# Autodesk Inventor assembly: KND-2000 Collector 01
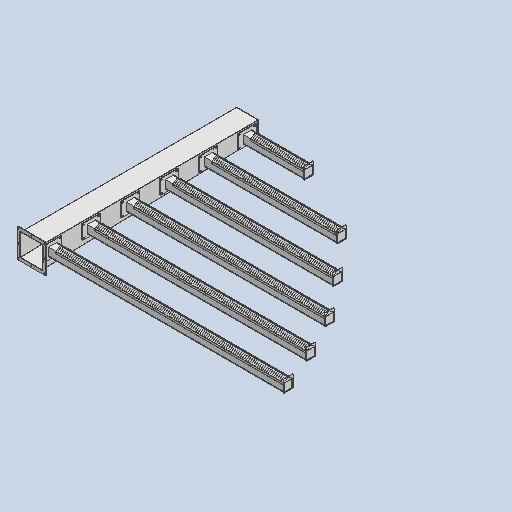
[picture p0: Inventor's stored thumbnail of the model, 512x512]
Saved by Autodesk Inventor 2026.2 (Build 302298000, 298)
## iProperties
Created: 2026-05-12
Part Number: KND-2000 Collector 01
Document SubType Name: Assembly
Designer: admin
Stock Number: Коллектор
Author: admin
## Documents named in this file (11)
- C:\Users\admin\Documents\Inventor\KND-DistribSystem\DRS_D1200\KND-2000 Collector 01.iam
- C:\Users\admin\Documents\Inventor\KND-DistribSystem\DRS_D1200\KND-1422 DrSysB diameter way up 01.ipt
- C:\Users\admin\Documents\Inventor\KND-DistribSystem\DRS_D1200\KND-1423 DrSysB diameter way down 01.ipt
- C:\Users\admin\Documents\Inventor\KND-DistribSystem\DRS_D1200\KND-1424 DrSysB diam way cup 01.ipt
- C:\Users\admin\Documents\Inventor\KND-DistribSystem\DRS_D1200\KND-1426 DrSysB Main way FLANGE 01.ipt
- C:\Users\admin\Documents\Inventor\KND-DistribSystem\DRS_D1200\KND-3100 Branch 1 01.iam
- C:\Users\admin\Documents\Inventor\KND-DistribSystem\DRS_D1200\KND-3200 Branch 2 01.iam
- C:\Users\admin\Documents\Inventor\KND-DistribSystem\DRS_D1200\KND-3300 Branch 3 01.iam
- C:\Users\admin\Documents\Inventor\KND-DistribSystem\DRS_D1200\KND-3400 Branch 4 01.iam
- C:\Users\admin\Documents\Inventor\KND-DistribSystem\DRS_D1200\KND-3500 Branch 5 01.iam
- C:\Users\admin\Documents\Inventor\KND-DistribSystem\DRS_D1200\KND-3600 Branch 6 01.iam
## Components (10 placed, 10 different names)
1. PRS 1422 DrSysB diameter way up_D1200:1 — Flush:10, Flush:9, Mate:11, Rigid:23, Mate:108
2. PRS 1423 DrSysB diameter way down_D1200:1 — Rigid:23, Mate:107, Flush:43, Mate:109, Mate:110, Mate:111, Mate:112, Mate:113, Mate:114, Mate:115, Mate:116, Mate:117, Mate:118, Mate:119, Mate:120, Mate:121, Mate:122, Mate:123, Mate:124, Mate:125, Mate:126
3. PRS 1424 DrSysB diam way cup_D1200:1 — Flush:10, Flush:9, Mate:11
4. KND-1426 DrSysB Main way FLANGE 01:1 — Mate:107, Mate:108, Flush:43
5. KND-3100 Branch 1 01:1 [sub-assembly] — Mate:109, Mate:110, Mate:111
6. KND-3200 Branch 2 01:1 [sub-assembly] — Mate:112, Mate:113, Mate:114
7. KND-3300 Branch 3 01:1 [sub-assembly] — Mate:115, Mate:116, Mate:117
8. KND-3400 Branch 4 01:1 [sub-assembly] — Mate:118, Mate:119, Mate:120
9. KND-3500 Branch 5 01:1 [sub-assembly] — Mate:121, Mate:122, Mate:123
10. KND-3600 Branch 6 01:1 [sub-assembly] — Mate:124, Mate:125, Mate:126
## Relationships (25: Mate 21, Flush 3, WeldJoint 1)
- Flush:10 (1 mm): PRS 1422 DrSysB diameter way up_D1200:1 ↔ PRS 1424 DrSysB diam way cup_D1200:1
- Flush:9 (-1 mm): PRS 1422 DrSysB diameter way up_D1200:1 ↔ PRS 1424 DrSysB diam way cup_D1200:1
- Mate:11: PRS 1422 DrSysB diameter way up_D1200:1 ↔ PRS 1424 DrSysB diam way cup_D1200:1
- Rigid:23 [WeldJoint]: PRS 1422 DrSysB diameter way up_D1200:1 ↔ PRS 1423 DrSysB diameter way down_D1200:1
- Mate:107 (1.1 mm): PRS 1423 DrSysB diameter way down_D1200:1 ↔ KND-1426 DrSysB Main way FLANGE 01:1
- Mate:108 (0.1 mm): PRS 1422 DrSysB diameter way up_D1200:1 ↔ KND-1426 DrSysB Main way FLANGE 01:1
- Flush:43: PRS 1423 DrSysB diameter way down_D1200:1 ↔ KND-1426 DrSysB Main way FLANGE 01:1
- Mate:109: PRS 1423 DrSysB diameter way down_D1200:1 ↔ KND-3100 Branch 1 01:1
- Mate:110 (0.25 mm): PRS 1423 DrSysB diameter way down_D1200:1 ↔ KND-3100 Branch 1 01:1
- Mate:111 (0.25 mm): PRS 1423 DrSysB diameter way down_D1200:1 ↔ KND-3100 Branch 1 01:1
- Mate:112: PRS 1423 DrSysB diameter way down_D1200:1 ↔ KND-3200 Branch 2 01:1
- Mate:113 (0.25 mm): PRS 1423 DrSysB diameter way down_D1200:1 ↔ KND-3200 Branch 2 01:1
- Mate:114 (0.25 mm): PRS 1423 DrSysB diameter way down_D1200:1 ↔ KND-3200 Branch 2 01:1
- Mate:115: PRS 1423 DrSysB diameter way down_D1200:1 ↔ KND-3300 Branch 3 01:1
- Mate:116 (0.25 mm): PRS 1423 DrSysB diameter way down_D1200:1 ↔ KND-3300 Branch 3 01:1
- Mate:117 (0.25 mm): PRS 1423 DrSysB diameter way down_D1200:1 ↔ KND-3300 Branch 3 01:1
- Mate:118: PRS 1423 DrSysB diameter way down_D1200:1 ↔ KND-3400 Branch 4 01:1
- Mate:119 (0.25 mm): PRS 1423 DrSysB diameter way down_D1200:1 ↔ KND-3400 Branch 4 01:1
- Mate:120 (0.25 mm): PRS 1423 DrSysB diameter way down_D1200:1 ↔ KND-3400 Branch 4 01:1
- Mate:121: PRS 1423 DrSysB diameter way down_D1200:1 ↔ KND-3500 Branch 5 01:1
- Mate:122 (0.25 mm): PRS 1423 DrSysB diameter way down_D1200:1 ↔ KND-3500 Branch 5 01:1
- Mate:123 (0.25 mm): PRS 1423 DrSysB diameter way down_D1200:1 ↔ KND-3500 Branch 5 01:1
- Mate:124: PRS 1423 DrSysB diameter way down_D1200:1 ↔ KND-3600 Branch 6 01:1
- Mate:125 (0.25 mm): PRS 1423 DrSysB diameter way down_D1200:1 ↔ KND-3600 Branch 6 01:1
- Mate:126 (0.25 mm): PRS 1423 DrSysB diameter way down_D1200:1 ↔ KND-3600 Branch 6 01:1
